# Autodesk Inventor assembly: CARRO ROBÓTICO
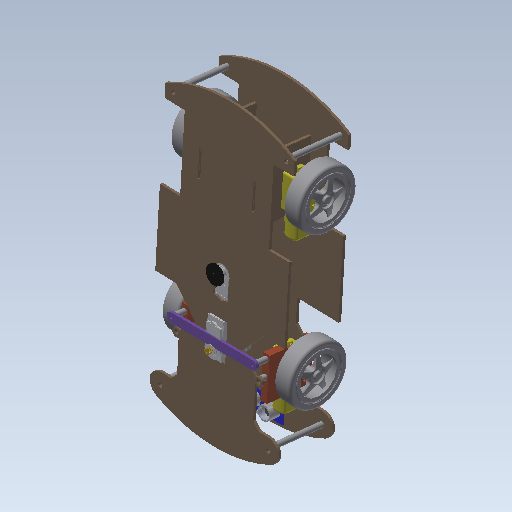
[picture p0: Inventor's stored thumbnail of the model, 512x512]
Saved by Autodesk Inventor 2021 (Build 250183000, 183)
## iProperties
Created: 2021-07-07
Part Number: CARRO ROBÓTICO
Document SubType Name: Assembly
Designer: Administrator
Mass: 616.366 g
Surface Area: 3427.79 cm^2
Volume: 616.366 cm^3
Density: 1 g/cm^3
Title: CARRO ROBÓTICO v2
Author: Administrator
## Documents named in this file (14)
- C:\Users\ASUS\Desktop\3d model\CARRO ROBÓTICO.iam
- C:\Users\ASUS\Desktop\3d model\Chassi.ipt
- C:\Users\ASUS\Desktop\3d model\SEPARADOR.ipt
- C:\Users\ASUS\Desktop\3d model\suporte traseiro.ipt
- C:\Users\ASUS\Desktop\3d model\Motor.ipt
- C:\Users\ASUS\Desktop\3d model\suporte traseiro_MIR.ipt
- C:\Users\ASUS\Desktop\3d model\Rad.ipt
- C:\Users\ASUS\Desktop\3d model\Chassi - Copia.ipt
- C:\Users\ASUS\Desktop\3d model\DIANTEIRA DIREITA.iam
- C:\Users\ASUS\Desktop\3d model\DIANTEIRA ESQUERDA.iam
- C:\Users\ASUS\Desktop\3d model\HASTE.ipt
- C:\Users\ASUS\Desktop\3d model\MG_996R (2).iam
- C:\Users\ASUS\Desktop\3d model\servo chih.ipt
- C:\Users\ASUS\Desktop\ul\ULTRASONIC SENSOR.ipt
## Components (19 placed, 13 different names)
1. Chassi:1 — Mate:1
2. SEPARADOR:1
3. SEPARADOR:2
4. SEPARADOR:3
5. SEPARADOR:4
6. suporte traseiro:1
7. Motor:3
8. Motor:4
9. suporte traseiro_MIR:1
10. Rad:3
11. Rad:4
12. Chassi - Copia:1
13. DIANTEIRA DIREITA:1 [sub-assembly]
14. DIANTEIRA ESQUERDA:1 [sub-assembly]
15. HASTE:1
16. MG_996R (2):3 [sub-assembly]
17. MG_996R (2):4 [sub-assembly]
18. servo chih:3
19. ULTRASONIC SENSOR:1 — Mate:1
## Relationships (1: Mate 1)
- Mate:1: Chassi:1 ↔ ULTRASONIC SENSOR:1
